# Autodesk Inventor assembly: x_axis
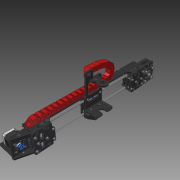
[picture p0: Inventor's stored thumbnail of the model, 180x180]
Saved by Autodesk Inventor 2014 (Build 180170000, 170)
## iProperties
Created: 2014-01-10
Part Number: x_axis
Document SubType Name: Assembly
Designer: buben
Author: buben
## Documents named in this file (12)
- C:\Users\buben\Documents\GitHub\bacon\inventor files\assemblies\x_axis.iam
- C:\Users\buben\Documents\GitHub\bacon\inventor files\assemblies\x_motor.iam
- C:\Users\buben\Documents\GitHub\bacon\inventor files\assemblies\x_iddler.iam
- C:\Users\buben\Documents\GitHub\bacon\inventor files\printer parts\x_axis_chain_holder.ipt
- C:\Users\buben\Documents\GitHub\bacon\inventor files\utils\x_axis_rod.ipt
- C:\Users\buben\Documents\GitHub\bacon\inventor files\assemblies\x_carryage.iam
- C:\Users\buben\Documents\GitHub\bacon\inventor files\utils\washer_m4.ipt
- C:\Users\buben\Documents\Inventor\Content Center Files\R2014\en-US\ISO 7040\ISO 7040 - M4.ipt
- C:\Users\buben\Documents\Inventor\Content Center Files\R2014\en-US\ISO 4762(2)\ISO 4762 - M4 x 30ISO.ipt
- C:\Users\buben\Documents\GitHub\bacon\inventor files\utils\x_axis_cable_mount_b.ipt
- C:\Users\buben\Documents\GitHub\bacon\inventor files\utils\cable_chain_22.ipt
- C:\Users\buben\Documents\GitHub\bacon\inventor files\utils\x_axis_cable_mount_a.ipt
## Components (47 placed, 11 different names)
1. x_motor:1 [sub-assembly] — Mate:1, Mate:2, Mate:3, Flush:1, Flush:2, Tangent:1, Tangent:2, Tangent:3, Tangent:4, Tangent:5, Tangent:6, Mate:4, Mate:5, Mate:6, Mate:17, Mate:18, Mate:19, Mate:20
2. x_iddler:1 [sub-assembly] — Flush:1, Flush:2, Tangent:7, Mate:21, Mate:22, Mate:23, Mate:24
3. x_axis_chain_holder:1 — Mate:4, Mate:5, Mate:6, Mate:9, Mate:10, Mate:11, Mate:12, Mate:13, Mate:14, Mate:15, Mate:16, Mate:37, Flush:4
4. x_axis_rod:1 — Tangent:2, Tangent:4, Tangent:5, Tangent:7, Mate:7
5. x_axis_rod:2 — Tangent:1, Tangent:3, Tangent:6, Mate:8
6. x_carryage:1 [sub-assembly] — Mate:7, Mate:8, Mate:34, Mate:38, Mate:39
7. CSN 02 1702 B B 4,3:1 — Mate:21, Mate:23, Mate:29
8. CSN 02 1702 B B 4,3:2 — Mate:19, Mate:20, Mate:25
9. CSN 02 1702 B B 4,3:3 — Mate:22, Mate:24, Mate:31
10. CSN 02 1702 B B 4,3:4 — Mate:17, Mate:18, Mate:27
11. CSN 02 1702 B B 4,3:5 — Mate:12, Mate:13, Insert:4
12. CSN 02 1702 B B 4,3:6 — Mate:11, Mate:14, Insert:3
13. CSN 02 1702 B B 4,3:7 — Mate:10, Mate:15, Insert:2
14. CSN 02 1702 B B 4,3:8 — Mate:9, Mate:16, Insert:1
15. ISO 4762 M4 x 30:2 — Insert:1, Mate:28
16. ISO 4762 M4 x 30:1 — Insert:2, Mate:26
17. ISO 4762 M4 x 30:4 — Insert:3, Mate:32
18. ISO 4762 M4 x 30:3 — Insert:4, Mate:30
19. DIN EN ISO 7040 M4:1 — Mate:31, Mate:32
20. DIN EN ISO 7040 M4:2 — Mate:29, Mate:30
21. DIN EN ISO 7040 M4:3 — Mate:27, Mate:28
22. DIN EN ISO 7040 M4:4 — Mate:25, Mate:26
23. x_axis_cable_mount_b:1 — Mate:34, Insert:52, Angle:48, Mate:38, Mate:39
24. cable_chain_22:26 — Insert:53, Flush:3
25. cable_chain_22:27
26. cable_chain_22:28
27. cable_chain_22:29
28. cable_chain_22:30
29. cable_chain_22:31
30. cable_chain_22:32
31. cable_chain_22:33
32. cable_chain_22:34
33. cable_chain_22:35
34. cable_chain_22:36
35. cable_chain_22:37
36. cable_chain_22:38
37. cable_chain_22:39
38. cable_chain_22:40
39. cable_chain_22:41
40. cable_chain_22:42
41. cable_chain_22:43
42. cable_chain_22:44
43. cable_chain_22:45
44. cable_chain_22:46
45. cable_chain_22:47
46. cable_chain_22:48 — Insert:52, Angle:48
47. x_axis_cable_mount_a:1 — Insert:53, Flush:3, Mate:37, Flush:4
## Relationships (98: Mate 36, Insert 28, Angle 23, Tangent 7, Flush 4)
- Mate:1: x_motor:1
- Mate:2: x_motor:1
- Mate:3: x_motor:1
- Flush:1: x_motor:1 ↔ x_iddler:1
- Flush:2: x_motor:1 ↔ x_iddler:1
- Tangent:1: x_motor:1 ↔ x_axis_rod:2
- Tangent:2: x_motor:1 ↔ x_axis_rod:1
- Tangent:3: x_motor:1 ↔ x_axis_rod:2
- Tangent:4: x_motor:1 ↔ x_axis_rod:1
- Tangent:5: x_motor:1 ↔ x_axis_rod:1
- Tangent:6: x_motor:1 ↔ x_axis_rod:2
- Tangent:7: x_iddler:1 ↔ x_axis_rod:1
- Mate:4: x_motor:1 ↔ x_axis_chain_holder:1
- Mate:5: x_motor:1 ↔ x_axis_chain_holder:1
- Mate:6: x_motor:1 ↔ x_axis_chain_holder:1
- Mate:7: x_axis_rod:1 ↔ x_carryage:1
- Mate:8: x_axis_rod:2 ↔ x_carryage:1
- Mate:9: x_axis_chain_holder:1 ↔ CSN 02 1702 B B 4,3:8
- Mate:10: x_axis_chain_holder:1 ↔ CSN 02 1702 B B 4,3:7
- Mate:11: x_axis_chain_holder:1 ↔ CSN 02 1702 B B 4,3:6
- Mate:12: x_axis_chain_holder:1 ↔ CSN 02 1702 B B 4,3:5
- Mate:13: x_axis_chain_holder:1 ↔ CSN 02 1702 B B 4,3:5
- Mate:14: x_axis_chain_holder:1 ↔ CSN 02 1702 B B 4,3:6
- Mate:15: x_axis_chain_holder:1 ↔ CSN 02 1702 B B 4,3:7
- Mate:16: x_axis_chain_holder:1 ↔ CSN 02 1702 B B 4,3:8
- Mate:17: x_motor:1 ↔ CSN 02 1702 B B 4,3:4
- Mate:18: x_motor:1 ↔ CSN 02 1702 B B 4,3:4
- Mate:19: x_motor:1 ↔ CSN 02 1702 B B 4,3:2
- Mate:20: x_motor:1 ↔ CSN 02 1702 B B 4,3:2
- Mate:21: x_iddler:1 ↔ CSN 02 1702 B B 4,3:1
- Mate:22: x_iddler:1 ↔ CSN 02 1702 B B 4,3:3
- Mate:23: x_iddler:1 ↔ CSN 02 1702 B B 4,3:1
- Mate:24: x_iddler:1 ↔ CSN 02 1702 B B 4,3:3
- Insert:1: CSN 02 1702 B B 4,3:8 ↔ ISO 4762 M4 x 30:2
- Insert:2: CSN 02 1702 B B 4,3:7 ↔ ISO 4762 M4 x 30:1
- Insert:3: CSN 02 1702 B B 4,3:6 ↔ ISO 4762 M4 x 30:4
- Insert:4: CSN 02 1702 B B 4,3:5 ↔ ISO 4762 M4 x 30:3
- Mate:25: CSN 02 1702 B B 4,3:2 ↔ DIN EN ISO 7040 M4:4
- Mate:26: ISO 4762 M4 x 30:1 ↔ DIN EN ISO 7040 M4:4
- Mate:27: CSN 02 1702 B B 4,3:4 ↔ DIN EN ISO 7040 M4:3
- Mate:28: ISO 4762 M4 x 30:2 ↔ DIN EN ISO 7040 M4:3
- Mate:29: CSN 02 1702 B B 4,3:1 ↔ DIN EN ISO 7040 M4:2
- Mate:30: ISO 4762 M4 x 30:3 ↔ DIN EN ISO 7040 M4:2
- Mate:31: CSN 02 1702 B B 4,3:3 ↔ DIN EN ISO 7040 M4:1
- Mate:32: ISO 4762 M4 x 30:4 ↔ DIN EN ISO 7040 M4:1
- Mate:34: x_carryage:1 ↔ x_axis_cable_mount_b:1
- [Insert]: cable_chain_22:26 ↔ cable_chain_22:27
- [Angle] (-36 deg): cable_chain_22:26 ↔ cable_chain_22:27
- [Insert]: cable_chain_22:28 ↔ cable_chain_22:29
- [Angle] (-36 deg): cable_chain_22:28 ↔ cable_chain_22:29
- [Insert]: cable_chain_22:29 ↔ cable_chain_22:30
- [Angle] (-36 deg): cable_chain_22:29 ↔ cable_chain_22:30
- [Insert]: cable_chain_22:27 ↔ cable_chain_22:28
- [Angle] (-36 deg): cable_chain_22:27 ↔ cable_chain_22:28
- [Insert]: cable_chain_22:31 ↔ cable_chain_22:32
- [Angle] (-36 deg): cable_chain_22:31 ↔ cable_chain_22:32
- [Insert]: cable_chain_22:32 ↔ cable_chain_22:33
- [Angle] (-36 deg): cable_chain_22:32 ↔ cable_chain_22:33
- [Insert]: cable_chain_22:34 ↔ cable_chain_22:35
- [Angle] (-36 deg): cable_chain_22:34 ↔ cable_chain_22:35
- [Insert]: cable_chain_22:35 ↔ cable_chain_22:36
- [Angle] (-36 deg): cable_chain_22:35 ↔ cable_chain_22:36
- [Insert]: cable_chain_22:33 ↔ cable_chain_22:34
- [Angle] (-36 deg): cable_chain_22:33 ↔ cable_chain_22:34
- [Insert]: cable_chain_22:30 ↔ cable_chain_22:31
- [Angle] (-36 deg): cable_chain_22:30 ↔ cable_chain_22:31
- [Insert]: cable_chain_22:37 ↔ cable_chain_22:38
- [Angle] (-36 deg): cable_chain_22:37 ↔ cable_chain_22:38
- [Insert]: cable_chain_22:38 ↔ cable_chain_22:39
- [Angle] (-36 deg): cable_chain_22:38 ↔ cable_chain_22:39
- [Insert]: cable_chain_22:40 ↔ cable_chain_22:41
- [Angle] (-36 deg): cable_chain_22:40 ↔ cable_chain_22:41
- [Insert]: cable_chain_22:41 ↔ cable_chain_22:42
- [Angle] (-36 deg): cable_chain_22:41 ↔ cable_chain_22:42
- [Insert]: cable_chain_22:39 ↔ cable_chain_22:40
- [Angle] (-36 deg): cable_chain_22:39 ↔ cable_chain_22:40
- [Insert]: cable_chain_22:43 ↔ cable_chain_22:44
- [Angle] (-36 deg): cable_chain_22:43 ↔ cable_chain_22:44
- [Insert]: cable_chain_22:44 ↔ cable_chain_22:45
- [Angle] (-36 deg): cable_chain_22:44 ↔ cable_chain_22:45
- [Insert]: cable_chain_22:46 ↔ cable_chain_22:47
- [Angle] (-36 deg): cable_chain_22:46 ↔ cable_chain_22:47
- [Insert]: cable_chain_22:47 ↔ cable_chain_22:48
- [Angle] (-36 deg): cable_chain_22:47 ↔ cable_chain_22:48
- [Insert]: cable_chain_22:45 ↔ cable_chain_22:46
- [Angle] (-36 deg): cable_chain_22:45 ↔ cable_chain_22:46
- [Insert]: cable_chain_22:42 ↔ cable_chain_22:43
- [Angle] (-36 deg): cable_chain_22:42 ↔ cable_chain_22:43
- [Insert]: cable_chain_22:36 ↔ cable_chain_22:37
- [Angle] (-36 deg): cable_chain_22:36 ↔ cable_chain_22:37
- Insert:52: x_axis_cable_mount_b:1 ↔ cable_chain_22:48
- Angle:48 (-36 deg): x_axis_cable_mount_b:1 ↔ cable_chain_22:48
- Insert:53: cable_chain_22:26 ↔ x_axis_cable_mount_a:1
- Flush:3: cable_chain_22:26 ↔ x_axis_cable_mount_a:1
- Mate:37: x_axis_chain_holder:1 ↔ x_axis_cable_mount_a:1
- Flush:4 (-5 mm): x_axis_chain_holder:1 ↔ x_axis_cable_mount_a:1
- Mate:38: x_carryage:1 ↔ x_axis_cable_mount_b:1
- Mate:39: x_carryage:1 ↔ x_axis_cable_mount_b:1
## Named parameters: d552_d406_d403 = -36 deg, d553_d407_d404 = 0 deg, d554_d408_d405 = -36 deg, d555_d409_d389 = -36 deg, d556_d410_d390 = 0 deg, d557_d411_d391 = -36 deg, d558_d412_d392_d389 = -36 deg, d559_d413_d393_d390 = 0 deg, d560_d414_d394_d391 = -36 deg, d561_d415_d395_d382 = 0 mm, d562_d416_d396_d383 = -36 deg, d563_d417_d397_d384 = 0 deg, d564_d418_d398_d385 = -36 deg, d565_d419_d399_d386 = 0 mm, d566_d420_d400_d387 = 0 mm, d567_d421_d401_d388 = 0 mm, d568_d422_d402 = 0 mm, d569_d423_d382 = 0 mm, d570_d424_d383 = -36 deg, d571_d425_d384 = 0 deg, d572_d426_d385 = -36 deg, d573_d427_d386 = 0 mm, d574_d428_d387 = 0 mm, d575_d429_d388 = 0 mm, d576_d430 = 0 mm, d577_d389 = -36 deg, d578_d390 = 0 deg, d579_d391 = -36 deg, d580_d392_d389 = -36 deg, d581_d393_d390 = 0 deg, d582_d394_d391 = -36 deg, d583_d395_d382 = 0 mm, d584_d396_d383 = -36 deg, d585_d397_d384 = 0 deg, d586_d398_d385 = -36 deg, d587_d399_d386 = 0 mm, d588_d400_d387 = 0 mm, d589_d401_d388 = 0 mm, d590_d402 = 0 mm, d595_d386 = 0 mm, d596_d387 = 0 mm, d597_d388 = 0 mm, d490_d486 = 0 mm, d491_d487 = -36 deg, d492_d488 = 0 deg, d493_d489 = -36 deg, d494_d431 = -36 deg, d495_d432 = 0 deg, d496_d433 = -36 deg, d497_d434_d431 = -36 deg, d498_d435_d432 = 0 deg, d499_d436_d433 = -36 deg, d500_d437_d403 = -36 deg, d501_d438_d404 = 0 deg, d502_d439_d405 = -36 deg, d503_d440_d406_d403 = -36 deg, d504_d441_d407_d404 = 0 deg, d505_d442_d408_d405 = -36 deg, d506_d443_d409_d389 = -36 deg, d507_d444_d410_d390 = 0 deg, d508_d445_d411_d391 = -36 deg, d509_d446_d412_d392_d389 = -36 deg, d510_d447_d413_d393_d390 = 0 deg, d511_d448_d414_d394_d391 = -36 deg, d512_d449_d415_d395_d382 = 0 mm, d513_d450_d416_d396_d383 = -36 deg, d514_d451_d417_d397_d384 = 0 deg, d515_d452_d418_d398_d385 = -36 deg, d516_d453_d419_d399_d386 = 0 mm, d517_d454_d420_d400_d387 = 0 mm, d518_d455_d421_d401_d388 = 0 mm, d519_d456_d422_d402 = 0 mm, d520_d457_d423_d382 = 0 mm, d521_d458_d424_d383 = -36 deg, d522_d459_d425_d384 = 0 deg, d523_d460_d426_d385 = -36 deg, d524_d461_d427_d386 = 0 mm, d525_d462_d428_d387 = 0 mm, d526_d463_d429_d388 = 0 mm, d527_d464_d430 = 0 mm, d528_d465_d389 = -36 deg, d529_d466_d390 = 0 deg, d530_d467_d391 = -36 deg, d531_d468_d392_d389 = -36 deg, d532_d469_d393_d390 = 0 deg, d533_d470_d394_d391 = -36 deg, d534_d471_d395_d382 = 0 mm, d535_d472_d396_d383 = -36 deg, d536_d473_d397_d384 = 0 deg, d537_d474_d398_d385 = -36 deg, d538_d475_d399_d386 = 0 mm, d539_d476_d400_d387 = 0 mm, d540_d477_d401_d388 = 0 mm, d541_d478_d402 = 0 mm, d542_d479_d382 = 0 mm, d543_d480_d383 = -36 deg, d544_d481_d384 = 0 deg, d545_d482_d385 = -36 deg, d546_d483_d386 = 0 mm, d547_d484_d387 = 0 mm, d548_d485_d388 = 0 mm, d549_d403 = -36 deg, d550_d404 = 0 deg, d551_d405 = -36 deg
